# Autodesk Inventor assembly: Assembly2
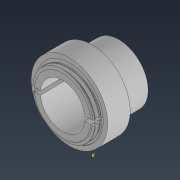
[picture p0: Inventor's stored thumbnail of the model, 180x180]
Saved by Autodesk Inventor 2022 (Build 260153000, 153)
## iProperties
Created: 2022-07-05
Part Number: Assembly2
Document SubType Name: Assembly
Designer: User
Author: User
## Documents named in this file (3)
- C:\Users\User\Documents\git\arduinomegashield\02_enclosure\Assembly2.iam
- C:\Users\User\Desktop\test_twist_friction_lock\bottomPiece2.ipt
- C:\Users\User\Documents\git\arduinomegashield\02_enclosure\topPiece2.ipt
## Components (2 placed, 2 different names)
1. bottomPiece2:1 — Mate:1
2. topPiece2:1 — Mate:1
## Relationships (1: Mate 1)
- Mate:1: bottomPiece2:1 ↔ topPiece2:1
